# Autodesk Inventor assembly: Robot Assembly 2
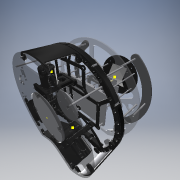
[picture p0: Inventor's stored thumbnail of the model, 180x180]
Saved by Autodesk Inventor 2018 (Build 220112000, 112)
## iProperties
Created: 2018-07-12
Part Number: Robot Assembly 2
Document SubType Name: Assembly
Designer: matth
Author: matth
## Documents named in this file (21)
- C:\Users\matth\Dropbox\M&A\Robotics-2018\Design and Hardware\Maxon Parts\Robot Assembly 2.iam
- C:\Users\matth\Dropbox\M&A\Robotics-2018\Design and Hardware\Maxon Parts\Base Plate.ipt
- C:\Users\matth\Dropbox\M&A\Robotics-2018\Design and Hardware\Maxon Parts\Capture Zone.ipt
- C:\Users\matth\Dropbox\M&A\Robotics-2018\Design and Hardware\Maxon Parts\Wheel Guard.ipt
- C:\Users\matth\Dropbox\M&A\Robotics-2018\Design and Hardware\Maxon Parts\Maxon Mount.ipt
- C:\Users\matth\Dropbox\M&A\Robotics-2018\Design and Hardware\Maxon Parts\50mm Standoff.ipt
- C:\Users\matth\Dropbox\M&A\Robotics-2018\Design and Hardware\Maxon Parts\TSSP Ring.ipt
- C:\Users\matth\Dropbox\M&A\Robotics-2018\Design and Hardware\Maxon Parts\40mm Standoff.ipt
- C:\Users\matth\Dropbox\M&A\Robotics-2018\Design and Hardware\Maxon Parts\Top Plate.ipt
- C:\Users\matth\Dropbox\M&A\Robotics-2018\Design and Hardware\Maxon Parts\10mm Standoff.ipt
- C:\Users\matth\Dropbox\M&A\Robotics-2018\Design and Hardware\Maxon Parts\Pixy Bracket.ipt
- C:\Users\matth\Dropbox\M&A\Robotics-2018\Design and Hardware\Maxon Parts\20mm Standoff.ipt
- C:\Users\matth\Dropbox\M&A\Robotics-2018\Design and Hardware\Maxon Parts\87.5mm Standoff.ipt
- C:\Users\matth\Dropbox\M&A\Robotics-2018\Design and Hardware\Maxon Parts\Mirror Mount.ipt
- C:\Users\matth\Dropbox\M&A\Robotics-2018\Design and Hardware\Maxon Parts\Pixy Sketch.ipt
- C:\Users\matth\Dropbox\M&A\Robotics-2018\Design and Hardware\Render Parts\TSSP Board.ipt
- C:\Users\matth\Dropbox\M&A\Robotics-2018\Design and Hardware\Render Parts\Light Sensor.ipt
- C:\Users\matth\Dropbox\M&A\Robotics-2018\Design and Hardware\Render Parts\TSSP Receiver.ipt
- C:\Users\matth\Dropbox\M&A\Robotics-2018\Design and Hardware\Render Parts\Teensy And Breakout.ipt
- C:\Users\matth\Dropbox\M&A\Robotics-2018\Design and Hardware\Render Parts\Power Supply.ipt
- C:\Users\matth\Dropbox\M&A\Robotics-2018\Design and Hardware\Maxon Parts\Arc.ipt
## Components (67 placed, 20 different names)
1. Capture Zone:1 — Mate:1
2. Base Plate:1 — Mate:1, Mate:2, Mate:3, Mate:4, Mate:5, Mate:6, Mate:7, Mate:8, Mate:9, Mate:10, Mate:11, Mate:12, Mate:13, Mate:14, Mate:66
3. Maxon Mount:1 — Mate:2
4. Maxon Mount:2 — Mate:5, Mate:6
5. Maxon Mount:3 — Mate:3, Mate:4
6. Wheel Guard:1 — Mate:7
7. Wheel Guard:2 — Mate:8, Mate:9, Mate:10
8. Wheel Guard:3 — Mate:11, Mate:12, Mate:15
9. 50mm Standoff:1 — Mate:14
10. 50mm Standoff:2 — Mate:13
11. TSSP Ring:1 — Mate:15, Mate:16, Mate:17, Mate:18, Mate:19, Mate:20, Mate:21, Mate:39, Mate:40, Mate:41, Mate:42, Mate:43, Mate:44, Mate:45, Mate:46, Mate:47, Mate:48, Mate:49, Mate:50, Mate:51, Mate:52, Mate:53, Mate:54, Mate:55, Mate:56, Mate:57, Mate:58, Mate:59, Mate:60, Mate:61, Mate:62, Mate:63, Mate:64, Mate:65, Mate:67, Mate:68, Mate:69, Mate:74, Mate:75, Mate:76, Mate:77
12. 40mm Standoff:1 — Mate:17
13. 40mm Standoff:2 — Mate:20
14. 40mm Standoff:3 — Mate:21
15. 40mm Standoff:4 — Mate:19
16. 40mm Standoff:5 — Mate:16
17. 40mm Standoff:6 — Mate:18, Mate:22
18. Top Plate:1 — Mate:22, Mate:23, Mate:24, Mate:25, Mate:26, Mate:79, Mate:80, Mate:81, Mate:82, Mate:85, Mate:86, Mate:87, Mate:88, Mate:92, Mate:93, Mate:100
19. 10mm Standoff:1 — Mate:26, Mate:27
20. 10mm Standoff:2 — Mate:25
21. 10mm Standoff:3 — Mate:24
22. 10mm Standoff:4 — Mate:23
23. Pixy Bracket:1 — Mate:27, Mate:96, Mate:97, Mate:98
24. Pixy Sketch:1 — Mate:99
25. 10mm Standoff:5 — Mate:39, Mate:72
26. 10mm Standoff:6 — Mate:40, Mate:73
27. 10mm Standoff:7 — Mate:41
28. 10mm Standoff:8 — Mate:42
29. TSSP Board:1 — Mate:58, Mate:59
30. TSSP Board:2 — Mate:62, Mate:63
31. TSSP Board:3 — Mate:54, Mate:55
32. TSSP Board:4 — Mate:64, Mate:65
33. TSSP Board:5 — Mate:43, Mate:44
34. TSSP Board:6 — Mate:47, Mate:48
35. TSSP Board:7 — Mate:45, Mate:46
36. TSSP Board:8 — Mate:49, Mate:50
37. TSSP Board:9 — Mate:51
38. TSSP Board:10 — Mate:52, Mate:53
39. TSSP Board:11 — Mate:60, Mate:61
40. TSSP Board:12 — Mate:56, Mate:57
41. Light Sensor:1 — Mate:66
42. 10mm Standoff:9 — Mate:67
43. 10mm Standoff:10 — Mate:69, Mate:71
44. 10mm Standoff:11 — Mate:68, Mate:70
45. TSSP Receiver:1 — Mate:70, Mate:71
46. Teensy And Breakout:1 — Mate:72, Mate:73
47. 10mm Standoff:12 — Mate:77
48. 10mm Standoff:13 — Mate:74, Mate:78
49. 10mm Standoff:14 — Mate:76
50. 10mm Standoff:15 — Mate:75
51. Power Supply:1 — Mate:78
52. 87.5mm Standoff:1 — Mate:79
53. 87.5mm Standoff:2 — Mate:80, Mate:94, Mate:100
54. 87.5mm Standoff:3 — Mate:81, Mate:95
55. 87.5mm Standoff:4 — Mate:82
56. 40mm Standoff:7 — Mate:85, Mate:89
57. 40mm Standoff:8 — Mate:86
58. 40mm Standoff:9 — Mate:87, Mate:91
59. 40mm Standoff:10 — Mate:88, Mate:90
60. Arc:1 — Mate:90, Mate:91
61. Arc:2 — Mate:89
62. 40mm Standoff:11 — Mate:92
63. 40mm Standoff:12 — Mate:93
64. Mirror Mount:1 — Mate:94, Mate:95
65. 20mm Standoff:1 — Mate:98
66. 20mm Standoff:2 — Mate:97
67. 20mm Standoff:3 — Mate:96, Mate:99
## Relationships (87: Mate 87)
- Mate:1: Capture Zone:1 ↔ Base Plate:1
- Mate:2: Base Plate:1 ↔ Maxon Mount:1
- Mate:3: Base Plate:1 ↔ Maxon Mount:3
- Mate:4: Base Plate:1 ↔ Maxon Mount:3
- Mate:5: Base Plate:1 ↔ Maxon Mount:2
- Mate:6: Base Plate:1 ↔ Maxon Mount:2
- Mate:7: Base Plate:1 ↔ Wheel Guard:1
- Mate:8: Base Plate:1 ↔ Wheel Guard:2
- Mate:9: Base Plate:1 ↔ Wheel Guard:2
- Mate:10: Base Plate:1 ↔ Wheel Guard:2
- Mate:11: Base Plate:1 ↔ Wheel Guard:3
- Mate:12: Base Plate:1 ↔ Wheel Guard:3
- Mate:13: Base Plate:1 ↔ 50mm Standoff:2
- Mate:14: Base Plate:1 ↔ 50mm Standoff:1
- Mate:15: Wheel Guard:3 ↔ TSSP Ring:1
- Mate:16: TSSP Ring:1 ↔ 40mm Standoff:5
- Mate:17: TSSP Ring:1 ↔ 40mm Standoff:1
- Mate:18: TSSP Ring:1 ↔ 40mm Standoff:6
- Mate:19: TSSP Ring:1 ↔ 40mm Standoff:4
- Mate:20: TSSP Ring:1 ↔ 40mm Standoff:2
- Mate:21: TSSP Ring:1 ↔ 40mm Standoff:3
- Mate:22: 40mm Standoff:6 ↔ Top Plate:1
- Mate:23: Top Plate:1 ↔ 10mm Standoff:4
- Mate:24: Top Plate:1 ↔ 10mm Standoff:3
- Mate:25: Top Plate:1 ↔ 10mm Standoff:2
- Mate:26: Top Plate:1 ↔ 10mm Standoff:1
- Mate:27: 10mm Standoff:1 ↔ Pixy Bracket:1
- Mate:39: TSSP Ring:1 ↔ 10mm Standoff:5
- Mate:40: TSSP Ring:1 ↔ 10mm Standoff:6
- Mate:41: TSSP Ring:1 ↔ 10mm Standoff:7
- Mate:42: TSSP Ring:1 ↔ 10mm Standoff:8
- Mate:43: TSSP Ring:1 ↔ TSSP Board:5
- Mate:44: TSSP Ring:1 ↔ TSSP Board:5
- Mate:45: TSSP Ring:1 ↔ TSSP Board:7
- Mate:46: TSSP Ring:1 ↔ TSSP Board:7
- Mate:47: TSSP Ring:1 ↔ TSSP Board:6
- Mate:48: TSSP Ring:1 ↔ TSSP Board:6
- Mate:49: TSSP Ring:1 ↔ TSSP Board:8
- Mate:50: TSSP Ring:1 ↔ TSSP Board:8
- Mate:51: TSSP Ring:1 ↔ TSSP Board:9
- Mate:52: TSSP Ring:1 ↔ TSSP Board:10
- Mate:53: TSSP Ring:1 ↔ TSSP Board:10
- Mate:54: TSSP Ring:1 ↔ TSSP Board:3
- Mate:55: TSSP Ring:1 ↔ TSSP Board:3
- Mate:56: TSSP Ring:1 ↔ TSSP Board:12
- Mate:57: TSSP Ring:1 ↔ TSSP Board:12
- Mate:58: TSSP Ring:1 ↔ TSSP Board:1
- Mate:59: TSSP Ring:1 ↔ TSSP Board:1
- Mate:60: TSSP Ring:1 ↔ TSSP Board:11
- Mate:61: TSSP Ring:1 ↔ TSSP Board:11
- Mate:62: TSSP Ring:1 ↔ TSSP Board:2
- Mate:63: TSSP Ring:1 ↔ TSSP Board:2
- Mate:64: TSSP Ring:1 ↔ TSSP Board:4
- Mate:65: TSSP Ring:1 ↔ TSSP Board:4
- Mate:66: Base Plate:1 ↔ Light Sensor:1
- Mate:67: TSSP Ring:1 ↔ 10mm Standoff:9
- Mate:68: TSSP Ring:1 ↔ 10mm Standoff:11
- Mate:69: TSSP Ring:1 ↔ 10mm Standoff:10
- Mate:70: 10mm Standoff:11 ↔ TSSP Receiver:1
- Mate:71: 10mm Standoff:10 ↔ TSSP Receiver:1
- Mate:72: 10mm Standoff:5 ↔ Teensy And Breakout:1
- Mate:73: 10mm Standoff:6 ↔ Teensy And Breakout:1
- Mate:74: TSSP Ring:1 ↔ 10mm Standoff:13
- Mate:75: TSSP Ring:1 ↔ 10mm Standoff:15
- Mate:76: TSSP Ring:1 ↔ 10mm Standoff:14
- Mate:77: TSSP Ring:1 ↔ 10mm Standoff:12
- Mate:78: 10mm Standoff:13 ↔ Power Supply:1
- Mate:79: Top Plate:1 ↔ 87.5mm Standoff:1
- Mate:80: Top Plate:1 ↔ 87.5mm Standoff:2
- Mate:81: Top Plate:1 ↔ 87.5mm Standoff:3
- Mate:82: Top Plate:1 ↔ 87.5mm Standoff:4
- Mate:85: Top Plate:1 ↔ 40mm Standoff:7
- Mate:86: Top Plate:1 ↔ 40mm Standoff:8
- Mate:87: Top Plate:1 ↔ 40mm Standoff:9
- Mate:88: Top Plate:1 ↔ 40mm Standoff:10
- Mate:89: 40mm Standoff:7 ↔ Arc:2
- Mate:90: 40mm Standoff:10 ↔ Arc:1
- Mate:91: 40mm Standoff:9 ↔ Arc:1
- Mate:92: Top Plate:1 ↔ 40mm Standoff:11
- Mate:93: Top Plate:1 ↔ 40mm Standoff:12
- Mate:94: 87.5mm Standoff:2 ↔ Mirror Mount:1
- Mate:95: 87.5mm Standoff:3 ↔ Mirror Mount:1
- Mate:96: Pixy Bracket:1 ↔ 20mm Standoff:3
- Mate:97: Pixy Bracket:1 ↔ 20mm Standoff:2
- Mate:98: Pixy Bracket:1 ↔ 20mm Standoff:1
- Mate:99: Pixy Sketch:1 ↔ 20mm Standoff:3
- Mate:100: Top Plate:1 ↔ 87.5mm Standoff:2
